# Autodesk Inventor assembly: BA1730
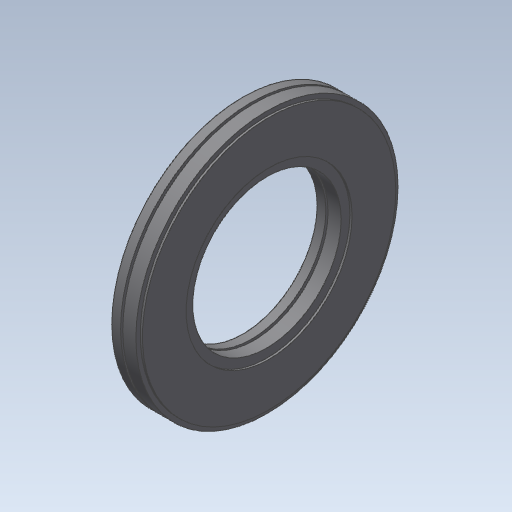
[picture p0: Inventor's stored thumbnail of the model, 512x512]
Saved by Autodesk Inventor 2024 (Build 280153000, 153)
## iProperties
Category: PARTsolutions
Company: MISUMI
Created: 2023-09-05
Part Number: BA1730
Catalog Web Link: www.cadenas.de
Description: BA_ _ _ _ _-Thrust Needle Roller Bearings with Retainers
Vendor: MISUMI
Document SubType Name: Assembly
Designer: psAdmin
Manufacturer: MISUMI
Mass: 1.86807 g
Surface Area: 34.7146 cm^2
Volume: 1.86807 cm^3
Density: 1 g/cm^3
PSOL_IDENT_0: {$CADENAS_DATA/23d-libs/misumi/metric/12_bearing_holders/ba1024_asmtab.prj},171 {VTYP=3D},{STYP=ASST
PSOL_IDENT_1: AB},{NB=BA1730},{LINA=BA1730},{NN=BA_ _ _ _ _},{DATE=03.06.2021 05:35:41},{GEOMDATE=19.10.2020 19:34
PSOL_IDENT_2: :04},{VERSION=},{LINEID=40},{WBVAR=},{WBNUMERIC=}  {NB=BA1730},{LINA=BA1730},{KT=DUMMY},{PN=BA1730},
PSOL_IDENT_3: {DD=17},{D=30},{B=2},{F=29.0},{F1=19.0},{DD1=17},{D1=30},{B1=1},{PPATH=ba1024_asmtpl.prj}
NB: BA1730
NN: BA_ _ _ _ _
NT: Thrust Needle Roller Bearings with Retainers
NBSYN: $PN.
LINA: BA1730
CATALOG: Misumi
PN: BA1730
DD: 17
D: 30
B: 2
F: 29
F1: 19
DD1: 17
D1: 30
B1: 1
SUPPLIER: MISUMI
ARTICLENO: BA1730
BOMINFO: BA1730
CREATOR: CADENAS GmbH
Title: BA1730
Author: Cadenas PARTsolutions
Comments: Thrust Needle Roller Bearings with Retainers
## Documents named in this file (3)
- C:\Users\michi\OneDrive - Kyoto University\lab\6_SHINOBI\FUHGA4\Design_Mechanism\5_birdeye\birdeye_shoulderUnit\_BA1730.iam
- C:\Users\michi\OneDrive - Kyoto University\lab\6_SHINOBI\FUHGA4\Design_Mechanism\5_birdeye\birdeye_shoulderUnit\BA1730_Autodesk_Inventor_2022_20230905\AIS2022\core_BA1730.ipt
- C:\Users\michi\OneDrive - Kyoto University\lab\6_SHINOBI\FUHGA4\Design_Mechanism\5_birdeye\birdeye_shoulderUnit\BA1730_Autodesk_Inventor_2022_20230905\AIS2022\washer_BA1730.ipt
## Components (3 placed, 2 different names)
1. core_BA1730:1 — core_to_washer_Z@1 <-> washer1_Z@2, core_to_washer_YZ@1 <-> washer1_YZ@2, core_to_washer1_XY@1 <-> washer2_XY@3, core_to_washer1_Z@1 <-> washer2_Z@3, core_to_washer1_YZ@1 <-> washer2_YZ@3
2. washer_BA1730:1 — core_to_washer_Z@1 <-> washer1_Z@2, core_to_washer_YZ@1 <-> washer1_YZ@2
3. washer_BA1730:2 — core_to_washer1_XY@1 <-> washer2_XY@3, core_to_washer1_Z@1 <-> washer2_Z@3, core_to_washer1_YZ@1 <-> washer2_YZ@3
## Relationships (5: Mate 3, Angle 2)
- core_to_washer_Z@1 <-> washer1_Z@2 [Mate]: core_BA1730:1 ↔ washer_BA1730:1
- core_to_washer_YZ@1 <-> washer1_YZ@2 [Angle] (0 deg): core_BA1730:1 ↔ washer_BA1730:1
- core_to_washer1_XY@1 <-> washer2_XY@3 [Mate] (1.5 mm): core_BA1730:1 ↔ washer_BA1730:2
- core_to_washer1_Z@1 <-> washer2_Z@3 [Mate]: core_BA1730:1 ↔ washer_BA1730:2
- core_to_washer1_YZ@1 <-> washer2_YZ@3 [Angle] (0 deg): core_BA1730:1 ↔ washer_BA1730:2
